# Autodesk Inventor assembly: Tread Sproket Gear Assembly
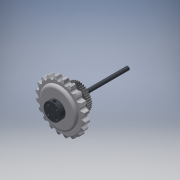
[picture p0: Inventor's stored thumbnail of the model, 180x180]
Saved by Autodesk Inventor 2016 (Build 200138000, 138)
## iProperties
Created: 2015-12-14
Part Number: Tread Sproket Gear Assembly
Document SubType Name: Assembly
Designer: tbloo
Author: tbloo
## Documents named in this file (6)
- C:\Users\tbloo\Documents\GitHub\phi_robotics\3d-models\FTC_Tetrix_KOP_Block_Party\Tim Bloot Designs\JAr JaR Bot\Tread Sproket Gear Assembly.iam
- C:\Users\tbloo\Documents\GitHub\phi_robotics\3d-models\FTC_Tetrix_KOP_Block_Party\Tetrix_Kit_FTC\Autodesk Inventor Files\tetrix_axle.ipt
- C:\Users\tbloo\Documents\GitHub\phi_robotics\3d-models\FTC_Tetrix_KOP_Block_Party\Tetrix_Kit_FTC\Autodesk Inventor Files\tetrix_bushing.ipt
- C:\Users\tbloo\Documents\GitHub\phi_robotics\3d-models\FTC_Tetrix_KOP_Block_Party\Tetrix_Kit_FTC\Autodesk Inventor Files\tetrix_tread_sprocket_2012.ipt
- C:\Users\tbloo\Documents\GitHub\phi_robotics\3d-models\FTC_Tetrix_KOP_Block_Party\Tetrix_Kit_FTC\Autodesk Inventor Files\tetrix_gear-small.ipt
- C:\Users\tbloo\Documents\GitHub\phi_robotics\3d-models\FTC_Tetrix_KOP_Block_Party\Tetrix_Kit_FTC\Autodesk Inventor Files\tetrix_axle_lock.iam
## Components (6 placed, 5 different names)
1. tetrix_axle:1 — Rigid:2
2. tetrix_tread_sprocket_2012:1 — Rotational:1, Rigid:1
3. tetrix_bushing:2 — Rotational:1, Rigid:4
4. tetrix_gear-small:1 — Rigid:3
5. tetrix_axle_lock:1 [sub-assembly] — Rigid:3, Rigid:4
6. tetrix_axle_lock:2 [sub-assembly] — Rigid:1, Rigid:2
## Relationships (5: WeldJoint 4, RevoluteJoint 1)
- Rotational:1 [RevoluteJoint]: tetrix_tread_sprocket_2012:1 ↔ tetrix_bushing:2
- Rigid:1 [WeldJoint]: tetrix_tread_sprocket_2012:1 ↔ tetrix_axle_lock:2
- Rigid:2 [WeldJoint]: tetrix_axle:1 ↔ tetrix_axle_lock:2
- Rigid:3 [WeldJoint]: tetrix_gear-small:1 ↔ tetrix_axle_lock:1
- Rigid:4 [WeldJoint]: tetrix_bushing:2 ↔ tetrix_axle_lock:1
